# Autodesk Inventor assembly: teljes3
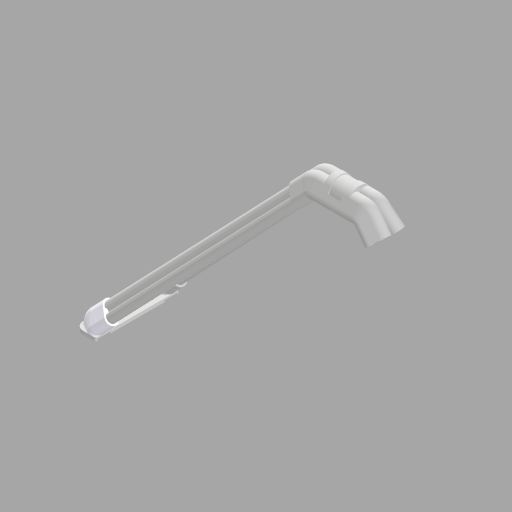
[picture p0: Inventor's stored thumbnail of the model, 512x512]
Saved by Autodesk Inventor 2023 (Build 270158000, 158)
## iProperties
Created: 2022-11-11
Part Number: teljes3
Document SubType Name: Assembly
Designer: gd1
Author: gd1
## Documents named in this file (5)
- C:\Users\gd1\3D Objects\3D nagyteherbírású híd\Híd\H-d\teljes7.iam
- C:\Users\gd1\3D Objects\3D nagyteherbírású híd\Híd\H-d\45 fok középre_talp2.ipt
- C:\Users\gd1\3D Objects\3D nagyteherbírású híd\Híd\H-d\palca 325mm.ipt
- C:\Users\gd1\3D Objects\3D nagyteherbírású híd\Híd\H-d\tipli.ipt
- C:\Users\gd1\3D Objects\3D nagyteherbírású híd\Híd\H-d\kozepcsati2.iam
## Components (6 placed, 4 different names)
1. 45 fok középre_talp2:1 — Rotational:1, Rotational:2, Rotational:3
2. palca 325mm:1 — Rotational:2, Rotational:3
3. palca 325mm:2 — Rotational:1, Rotational:4
4. tipli:1
5. tipli:2
6. kozepcsati2:1 [sub-assembly] — Rotational:4
## Relationships (4: RevoluteJoint 4)
- Rotational:1 [RevoluteJoint]: 45 fok középre_talp2:1 ↔ palca 325mm:2
- Rotational:2 [RevoluteJoint]: 45 fok középre_talp2:1 ↔ palca 325mm:1
- Rotational:3 [RevoluteJoint]: 45 fok középre_talp2:1 ↔ palca 325mm:1
- Rotational:4 [RevoluteJoint]: palca 325mm:2 ↔ kozepcsati2:1
